# Autodesk Inventor assembly: ServoMotor_CaseTH
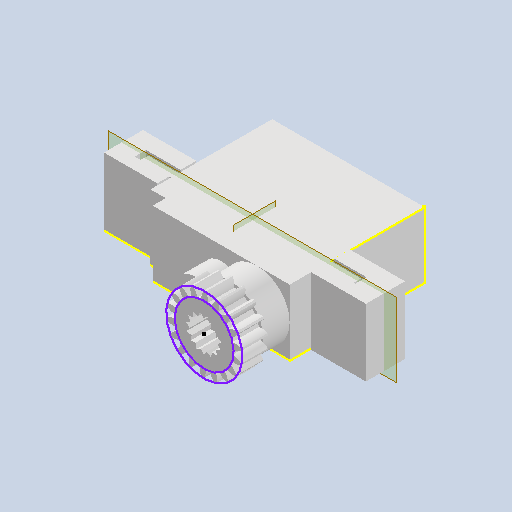
[picture p0: Inventor's stored thumbnail of the model, 512x512]
Saved by Autodesk Inventor 2024 (Build 280153000, 153)
## iProperties
Created: 2023-10-03
Part Number: ServoMotor_CaseTH
Document SubType Name: Assembly
Designer: Alexander Saavedra
Author: Alexander Saavedra
## Documents named in this file (4)
- D:\OneDrive - Escuela Politécnica Nacional\Documentos\Estudios\Escuela Politecnica Nacional\5to Semestre\Laboratorio IA y ML\Repositorios\Mano Derecha Custom\Mechanic Design\Motor Case\servoMotor\ServoMotor_CaseTH.iam
- D:\OneDrive - Escuela Politécnica Nacional\Documentos\Estudios\Escuela Politecnica Nacional\5to Semestre\Laboratorio IA y ML\Repositorios\Mano Derecha Custom\Mechanic Design\Motor Case\servoMotor\Servo.ipt
- D:\OneDrive - Escuela Politécnica Nacional\Documentos\Estudios\Escuela Politecnica Nacional\5to Semestre\Laboratorio IA y ML\Repositorios\Mano Derecha Custom\Mechanic Design\Motor Case\servoMotor\Servo Spur Gea.ipt
- D:\OneDrive - Escuela Politécnica Nacional\Documentos\Estudios\Escuela Politecnica Nacional\5to Semestre\Laboratorio IA y ML\Repositorios\Mano Derecha Custom\Mechanic Design\Motor Case\servoMotor Case\porta servo EPN v2 TH.ipt
## Components (3 placed, 3 different names)
1. Servo:1 — Rotational:1, Mate:2, Mate:3, Flush:1
2. Servo Spur Gea:1 — Rotational:1
3. porta servo EPN v2 TH:1 — Mate:2, Mate:3, Flush:1
## Relationships (4: Mate 2, RevoluteJoint 1, Flush 1)
- Rotational:1 [RevoluteJoint]: Servo:1 ↔ Servo Spur Gea:1
- Mate:2: Servo:1 ↔ porta servo EPN v2 TH:1
- Mate:3: Servo:1 ↔ porta servo EPN v2 TH:1
- Flush:1: Servo:1 ↔ porta servo EPN v2 TH:1
